# Autodesk Inventor assembly: omuniwheel
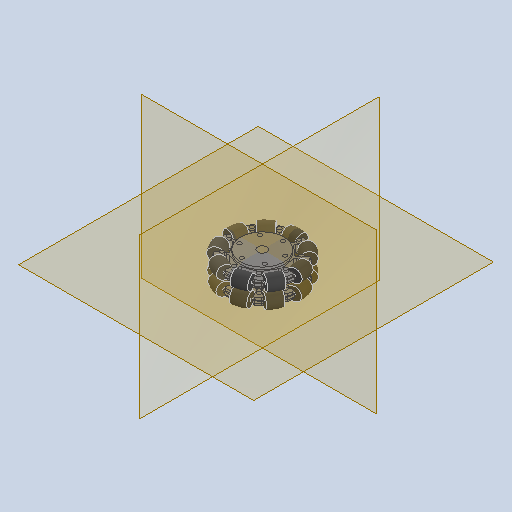
[picture p0: Inventor's stored thumbnail of the model, 512x512]
Saved by Autodesk Inventor 2025.2 (Build 292293000, 293)
## iProperties
Created: 2023-11-21
Part Number: omuniwheel
Document SubType Name: Assembly
Designer: haruy
Mass: 543.631 g
Surface Area: 679.733 cm^2
Volume: 146.025 cm^3
Density: 3.72287 g/cm^3
Author: fhbdh
## Documents named in this file (6)
- C:\Users\haruy\Documents\ロボコン\NHK2025\cad\nagahisa\gazebo\omuniwheel.iam
- C:\Users\haruy\Documents\ロボコン\NHK2025\cad\nagahisa\base_weel\takagi_weel\Workspaces\作業スペース\takagi\omuni_wheel_ver2.0\parts\frequently used parts\タイヤ\omni wheel\100mm wheel\omuni_flame_MIR1.ipt
- C:\Users\haruy\Documents\ロボコン\NHK2025\cad\nagahisa\base_weel\takagi_weel\Workspaces\作業スペース\takagi\omuni_wheel_ver2.0\parts\frequently used parts\タイヤ\omni wheel\100mm wheel\omuni_rubber_MIR1.ipt
- C:\Users\haruy\Documents\ロボコン\NHK2025\cad\nagahisa\base_weel\takagi_weel\Workspaces\作業スペース\takagi\omuni_wheel_ver2.0\parts\frequently used parts\タイヤ\omni wheel\100mm wheel\frange_MIR1.ipt
- C:\Users\haruy\Documents\ロボコン\NHK2025\cad\nagahisa\base_weel\takagi_weel\Workspaces\作業スペース\takagi\omuni_wheel_ver2.0\parts\frequently used parts\タイヤ\omni wheel\100mm wheel\al_shaft_MIR1.ipt
- C:\Users\haruy\Documents\ロボコン\NHK2025\cad\nagahisa\base_weel\takagi_weel\Workspaces\作業スペース\takagi\omuni_wheel_ver2.0\parts\frequently used parts\タイヤ\omni wheel\100mm wheel\nut_MIR1.ipt
## Components (27 placed, 5 different names)
1. omuni_flame_MIR1:1 — 挿入:3, 挿入:4, 挿入:5, 挿入:9, 挿入:8, 挿入:7, 挿入:2, 挿入:6, 挿入:1, メイト:1, 挿入:19, 挿入:22, 挿入:21, 挿入:20
2. omuni_rubber_MIR1:1 — 挿入:3
3. omuni_rubber_MIR1:2 — 挿入:4
4. omuni_rubber_MIR1:3 — 挿入:5
5. omuni_rubber_MIR1:4 — 挿入:9
6. omuni_rubber_MIR1:5 — 挿入:8
7. omuni_rubber_MIR1:6 — 挿入:7
8. omuni_rubber_MIR1:7 — 挿入:2
9. omuni_rubber_MIR1:8 — 挿入:6
10. omuni_rubber_MIR1:9 — メイト:3, 挿入:1
11. frange_MIR1:1 — メイト:1, 挿入:19, フラッシュ:3, 正接:1
12. omuni_flame_MIR1:2 — 挿入:25, 挿入:26, 挿入:27, 挿入:28, 挿入:29, 挿入:30
13. al_shaft_MIR1:1 — 挿入:22, 挿入:25
14. al_shaft_MIR1:2 — 挿入:21, 挿入:26
15. al_shaft_MIR1:3 — 挿入:20
16. nut_MIR1:1 — 挿入:27
17. nut_MIR1:2 — 挿入:28
18. nut_MIR1:3 — 挿入:29
19. omuni_rubber_MIR1:12 — 挿入:30
20. omuni_rubber_MIR1:13
21. omuni_rubber_MIR1:14
22. omuni_rubber_MIR1:15
23. omuni_rubber_MIR1:16
24. omuni_rubber_MIR1:17
25. omuni_rubber_MIR1:18
26. omuni_rubber_MIR1:19
27. omuni_rubber_MIR1:20
## Component patterns: (9 elements, first: omuni_rubber_MIR1:12)
## Relationships (25: Insert 19, Flush 2, Mate 2, Angle 1, Tangent 1)
- 挿入:3 [Insert]: omuni_flame_MIR1:1 ↔ omuni_rubber_MIR1:1
- 挿入:4 [Insert]: omuni_flame_MIR1:1 ↔ omuni_rubber_MIR1:2
- 挿入:5 [Insert]: omuni_flame_MIR1:1 ↔ omuni_rubber_MIR1:3
- 挿入:9 [Insert]: omuni_flame_MIR1:1 ↔ omuni_rubber_MIR1:4
- 挿入:8 [Insert]: omuni_flame_MIR1:1 ↔ omuni_rubber_MIR1:5
- 挿入:7 [Insert]: omuni_flame_MIR1:1 ↔ omuni_rubber_MIR1:6
- 挿入:2 [Insert]: omuni_flame_MIR1:1 ↔ omuni_rubber_MIR1:7
- 挿入:6 [Insert]: omuni_flame_MIR1:1 ↔ omuni_rubber_MIR1:8
- メイト:3 [Flush]: omuni_rubber_MIR1:9
- 挿入:1 [Insert]: omuni_flame_MIR1:1 ↔ omuni_rubber_MIR1:9
- メイト:1 [Mate]: omuni_flame_MIR1:1 ↔ frange_MIR1:1
- 挿入:19 [Insert]: omuni_flame_MIR1:1 ↔ frange_MIR1:1
- 挿入:22 [Insert]: omuni_flame_MIR1:1 ↔ al_shaft_MIR1:1
- 挿入:21 [Insert]: omuni_flame_MIR1:1 ↔ al_shaft_MIR1:2
- 挿入:20 [Insert]: omuni_flame_MIR1:1 ↔ al_shaft_MIR1:3
- フラッシュ:3 [Flush] (16 mm): frange_MIR1:1
- 角度:1 [Angle] (0 deg)
- 正接:1 [Tangent]: frange_MIR1:1
- メイト:2 [Mate] (12 mm)
- 挿入:25 [Insert]: omuni_flame_MIR1:2 ↔ al_shaft_MIR1:1
- 挿入:26 [Insert]: omuni_flame_MIR1:2 ↔ al_shaft_MIR1:2
- 挿入:27 [Insert]: omuni_flame_MIR1:2 ↔ nut_MIR1:1
- 挿入:28 [Insert]: omuni_flame_MIR1:2 ↔ nut_MIR1:2
- 挿入:29 [Insert]: omuni_flame_MIR1:2 ↔ nut_MIR1:3
- 挿入:30 [Insert]: omuni_flame_MIR1:2 ↔ omuni_rubber_MIR1:12
